# Autodesk Inventor assembly: Assembly
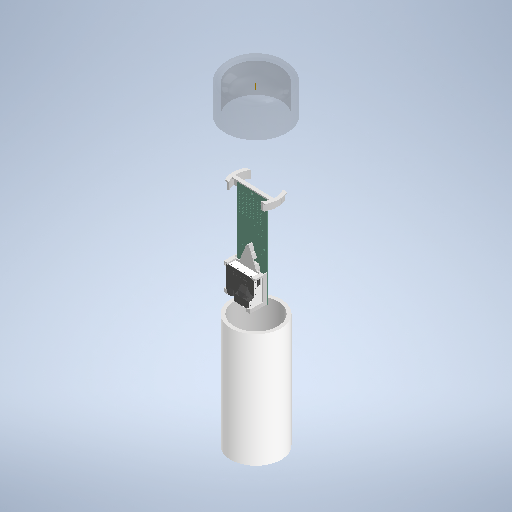
[picture p0: Inventor's stored thumbnail of the model, 512x512]
Saved by Autodesk Inventor 2025 (Build 290162010, 162A)
## iProperties
Created: 2024-06-25
Part Number: Assembly
Document SubType Name: Assembly
Designer: vncnt
Author: vncnt
## Documents named in this file (7)
- C:\Users\vncnt\Documents\GitHub\Air-Quality-Sensor\AQS-Mount\Assembly.iam
- C:\Users\vncnt\Documents\GitHub\Air-Quality-Sensor\AQS-Mount\AQS_Mount.ipt
- C:\Users\vncnt\Documents\GitHub\Air-Quality-Sensor\AQS-Mount\PVC.ipt
- C:\Users\vncnt\Documents\GitHub\Air-Quality-Sensor\AQS-Mount\SEN5X_Mount.ipt
- C:\Users\vncnt\Documents\GitHub\Air-Quality-Sensor\AQS-Mount\CSL_AQS_V1_spin3.iam
- C:\Users\vncnt\Documents\GitHub\Air-Quality-Sensor\AQS-Mount\Sensirion_STEP_SEN5x\Sensirion_STEP_SEN5x.ipt
- C:\Users\vncnt\Documents\GitHub\Air-Quality-Sensor\AQS-Mount\3in End Cap\3in End Cap.ipt
## Components (6 placed, 6 different names)
1. AQS_Mount:1 — Mate:6, Mate:11, Flush:1, Mate:13
2. CSL_AQS_V1_spin3:1 [sub-assembly] — Mate:6, Mate:9, Mate:13, Mate:14
3. SEN5X_Mount:1 — Mate:7, Mate:8, Mate:9, Mate:10, Mate:14
4. Sensirion_STEP_SEN5x:1 — Mate:7, Mate:8, Mate:10
5. 3in End Cap:1 — Mate:12
6. PVC:1 — Mate:11, Flush:1, Mate:12
## Relationships (10: Mate 9, Flush 1)
- Mate:6: AQS_Mount:1 ↔ CSL_AQS_V1_spin3:1
- Mate:7: SEN5X_Mount:1 ↔ Sensirion_STEP_SEN5x:1
- Mate:8: SEN5X_Mount:1 ↔ Sensirion_STEP_SEN5x:1
- Mate:9: CSL_AQS_V1_spin3:1 ↔ SEN5X_Mount:1
- Mate:10: SEN5X_Mount:1 ↔ Sensirion_STEP_SEN5x:1
- Mate:11: AQS_Mount:1 ↔ PVC:1
- Flush:1: AQS_Mount:1 ↔ PVC:1
- Mate:12: 3in End Cap:1 ↔ PVC:1
- Mate:13: AQS_Mount:1 ↔ CSL_AQS_V1_spin3:1
- Mate:14: CSL_AQS_V1_spin3:1 ↔ SEN5X_Mount:1
## Named parameters: Finish1_Area = 296.554, Finish2_Area = 571.981
note: some values were not read from the file. Shown as the stored number, unit unknown: "Finish1_Area", "Finish2_Area".
